# Autodesk Inventor assembly: FULL
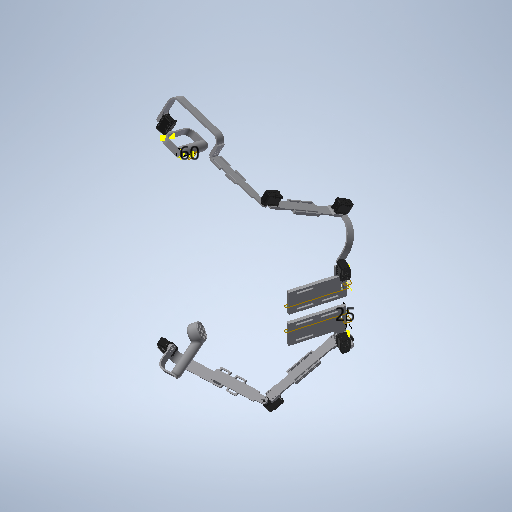
[picture p0: Inventor's stored thumbnail of the model, 512x512]
Saved by Autodesk Inventor 2025.1 (Build 291241000, 241)
## iProperties
Created: 2018-10-23
Part Number: FULL
Material: 일반
Document SubType Name: Assembly
Designer: otm09
Author: otm09
## Documents named in this file (15)
- C:\Users\goode\OneDrive\바탕 화면\3d 설계\3D Design\FULL.iam
- C:\Users\goode\OneDrive\바탕 화면\3d 설계\3D Design\arm1.ipt
- C:\Users\goode\OneDrive\바탕 화면\3d 설계\3D Design\AX-12.iam
- C:\Users\goode\OneDrive\바탕 화면\3d 설계\3D Design\shoulder1.ipt
- C:\Users\goode\OneDrive\바탕 화면\3d 설계\3D Design\shoulder2.ipt
- C:\Users\goode\OneDrive\바탕 화면\3d 설계\3D Design\hand_joy.ipt
- C:\Users\goode\OneDrive\바탕 화면\3d 설계\3D Design\hand_joy_cover.ipt
- C:\Users\goode\OneDrive\바탕 화면\3d 설계\3D Design\hand.ipt
- C:\Users\goode\OneDrive\바탕 화면\3d 설계\3D Design\hand-1.ipt
- C:\Users\goode\OneDrive\바탕 화면\3d 설계\3D Design\arm1_MIR.ipt
- C:\Users\goode\OneDrive\바탕 화면\3d 설계\3D Design\shoulder1_MIR.ipt
- C:\Users\goode\OneDrive\바탕 화면\3d 설계\3D Design\shoulder2_MIR.ipt
- C:\Users\goode\OneDrive\바탕 화면\3d 설계\3D Design\hand_MIR.ipt
- C:\Users\goode\OneDrive\바탕 화면\3d 설계\3D Design\hand-1_MIR.ipt
- C:\Users\goode\OneDrive\바탕 화면\3d 설계\3D Design\hand_joy_left_v2.ipt
## Components (23 placed, 14 different names)
1. arm1:1 — 강체:2, 강체:7
2. AX-12:1 [sub-assembly] — 강체:7, 회전:7
3. shoulder1:1 — 강체:8
4. AX-12:2 [sub-assembly] — 강체:8, 회전:3
5. arm1:2 — 강체:1, 강체:2
6. shoulder2:1 — 회전:3, 회전:4
7. AX-12:3 [sub-assembly] — 회전:4, 강체:1
8. hand_joy:1 — 회전:6, 강체:11
9. hand_joy_cover:1 — 강체:11
10. AX-12:4 [sub-assembly] — 회전:6, 강체:14
11. hand:1 — 강체:12, 회전:7
12. hand-1:1 — 강체:12, 강체:14
13. arm1_MIR:1 — 강체:15, 강체:17
14. AX-12:5 [sub-assembly] — 강체:15, 회전:10
15. shoulder1_MIR:1 — 강체:16
16. AX-12:6 [sub-assembly] — 강체:16, 회전:8
17. arm1_MIR:2 — 강체:17, 강체:18
18. shoulder2_MIR:1 — 회전:8, 회전:9
19. AX-12:7 [sub-assembly] — 회전:9, 강체:18
20. AX-12:8 [sub-assembly] — 강체:19, 회전:11, 회전:12
21. hand_MIR:1 — 회전:10, 강체:20
22. hand-1_MIR:1 — 강체:19, 강체:20
23. hand_joy_left_v2:1 — 회전:11, 회전:12
## Relationships (22: WeldJoint 13, RevoluteJoint 9)
- 강체:8 [WeldJoint]: shoulder1:1 ↔ AX-12:2
- 회전:3 [RevoluteJoint]: AX-12:2 ↔ shoulder2:1
- 회전:4 [RevoluteJoint]: shoulder2:1 ↔ AX-12:3
- 강체:1 [WeldJoint]: arm1:2 ↔ AX-12:3
- 강체:2 [WeldJoint]: arm1:1 ↔ arm1:2
- 강체:7 [WeldJoint]: arm1:1 ↔ AX-12:1
- 회전:6 [RevoluteJoint]: hand_joy:1 ↔ AX-12:4
- 강체:11 [WeldJoint]: hand_joy:1 ↔ hand_joy_cover:1
- 강체:12 [WeldJoint]: hand:1 ↔ hand-1:1
- 강체:14 [WeldJoint]: AX-12:4 ↔ hand-1:1
- 회전:7 [RevoluteJoint]: AX-12:1 ↔ hand:1
- 강체:15 [WeldJoint]: arm1_MIR:1 ↔ AX-12:5
- 강체:16 [WeldJoint]: shoulder1_MIR:1 ↔ AX-12:6
- 강체:17 [WeldJoint]: arm1_MIR:1 ↔ arm1_MIR:2
- 회전:8 [RevoluteJoint]: AX-12:6 ↔ shoulder2_MIR:1
- 회전:9 [RevoluteJoint]: shoulder2_MIR:1 ↔ AX-12:7
- 강체:18 [WeldJoint]: arm1_MIR:2 ↔ AX-12:7
- 회전:10 [RevoluteJoint]: AX-12:5 ↔ hand_MIR:1
- 강체:19 [WeldJoint]: AX-12:8 ↔ hand-1_MIR:1
- 강체:20 [WeldJoint]: hand_MIR:1 ↔ hand-1_MIR:1
- 회전:11 [RevoluteJoint]: AX-12:8 ↔ hand_joy_left_v2:1
- 회전:12 [RevoluteJoint]: AX-12:8 ↔ hand_joy_left_v2:1
